# Autodesk Inventor assembly: 惯性筛偏心轮装配
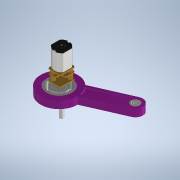
[picture p0: Inventor's stored thumbnail of the model, 180x180]
Saved by Autodesk Inventor 2022 (Build 260153000, 153)
## iProperties
Created: 2022-05-21
Part Number: 惯性筛偏心轮装配
Document SubType Name: Assembly
Designer: zhcne
Author: zhcne
## Documents named in this file (8)
- E:\Engineering_Development\SchoolProjects\2022_5_18_惯性筛_机电一体化课程设计\inertiascreen_curriculumdesign\3.Model\2.3D_Simulation\惯性筛偏心轮装配.iam
- E:\Engineering_Development\SchoolProjects\2022_5_18_惯性筛_机电一体化课程设计\inertiascreen_curriculumdesign\3.Model\2.3D_Simulation\Ipt\1.偏心轮\偏心轮.ipt
- E:\Engineering_Development\SchoolProjects\2022_5_18_惯性筛_机电一体化课程设计\inertiascreen_curriculumdesign\3.Model\2.3D_Simulation\Ipt\1.偏心轮\偏心轮外连接件.ipt
- C:\Users\zhcne\Documents\Inventor\Content Center Files\R2022\zh-CN\UNI ISO 1224 M\ISO 1224 - 38 3 x  7 x  3.ipt
- C:\Users\zhcne\Documents\Inventor\Content Center Files\R2022\zh-CN\UNI ISO 1224 M\ISO 1224 - 19 9 x  20 x  6.ipt
- C:\Users\zhcne\Documents\Inventor\Content Center Files\R2022\zh-CN\UNI ISO 1224 M\ISO 1224 - 19 2.5 x  7 x  2.5.ipt
- E:\Engineering_Development\SchoolProjects\2022_5_18_惯性筛_机电一体化课程设计\inertiascreen_curriculumdesign\3.Model\2.3D_Simulation\Ipt\1.偏心轮\GA12-N20微型减速直流电机3V_15RPM_8mm.iam
- E:\Engineering_Development\SchoolProjects\2022_5_18_惯性筛_机电一体化课程设计\inertiascreen_curriculumdesign\3.Model\2.3D_Simulation\Ipt\1.偏心轮\偏心支轴.ipt
## Components (8 placed, 7 different names)
1. GA12-N20微型减速直流电机3V_15RPM_8mm:1 [sub-assembly] — 配合:8, 配合:10, 配合:13, 配合:15
2. 偏心轮:1 — 插入:2, 配合:2, 表面齐平:1, 配合:8, 配合:10, 配合:11, 配合:15
3. 偏心轮外连接件:1 — 配合:2, 表面齐平:1, 配合:3, 配合:4, 配合:5, 配合:6, 配合:14, 表面齐平:2
4. UNI ISO 1224 (mm) 38 3 x  7 x  3:1 — 插入:2, 配合:12
5. UNI ISO 1224 (mm) 19 9 x  20 x  6:1 — 配合:3, 配合:4
6. UNI ISO 1224 (mm) 19 2.5 x  7 x  2.5:1 — 配合:5, 配合:6
7. UNI ISO 1224 (mm) 19 2.5 x  7 x  2.5:2 — 配合:14, 表面齐平:2
8. 偏心支轴:1 — 配合:11, 配合:12, 配合:13
## Relationships (15: Mate 12, Flush 2, Insert 1)
- 插入:2 [Insert]: 偏心轮:1 ↔ UNI ISO 1224 (mm) 38 3 x  7 x  3:1
- 配合:2 [Mate]: 偏心轮:1 ↔ 偏心轮外连接件:1
- 表面齐平:1 [Flush]: 偏心轮:1 ↔ 偏心轮外连接件:1
- 配合:3 [Mate]: 偏心轮外连接件:1 ↔ UNI ISO 1224 (mm) 19 9 x  20 x  6:1
- 配合:4 [Mate]: 偏心轮外连接件:1 ↔ UNI ISO 1224 (mm) 19 9 x  20 x  6:1
- 配合:5 [Mate]: 偏心轮外连接件:1 ↔ UNI ISO 1224 (mm) 19 2.5 x  7 x  2.5:1
- 配合:6 [Mate]: 偏心轮外连接件:1 ↔ UNI ISO 1224 (mm) 19 2.5 x  7 x  2.5:1
- 配合:8 [Mate]: GA12-N20微型减速直流电机3V_15RPM_8mm:1 ↔ 偏心轮:1
- 配合:10 [Mate]: GA12-N20微型减速直流电机3V_15RPM_8mm:1 ↔ 偏心轮:1
- 配合:11 [Mate]: 偏心轮:1 ↔ 偏心支轴:1
- 配合:12 [Mate]: UNI ISO 1224 (mm) 38 3 x  7 x  3:1 ↔ 偏心支轴:1
- 配合:13 [Mate]: GA12-N20微型减速直流电机3V_15RPM_8mm:1 ↔ 偏心支轴:1
- 配合:14 [Mate]: 偏心轮外连接件:1 ↔ UNI ISO 1224 (mm) 19 2.5 x  7 x  2.5:2
- 表面齐平:2 [Flush]: 偏心轮外连接件:1 ↔ UNI ISO 1224 (mm) 19 2.5 x  7 x  2.5:2
- 配合:15 [Mate] (0.3 mm): GA12-N20微型减速直流电机3V_15RPM_8mm:1 ↔ 偏心轮:1
